# Autodesk Inventor assembly: Upper Lift Limit Switch
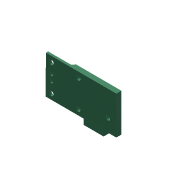
[picture p0: Inventor's stored thumbnail of the model, 180x180]
Saved by Autodesk Inventor 2018 (Build 220112000, 112)
## iProperties
Created: 2018-12-23
Part Number: Upper Lift Limit Switch
Document SubType Name: Assembly
Designer: ball
Author: ball
## Documents named in this file (3)
- C:\FTC\FTC8863CAD\2018Robot\Upper Lift Limit Switch.iam
- C:\FTC\FTC8863CAD\2018Robot\VWheelArmThickRIght.ipt
- C:\FTC\FTC8863CAD\Actobotics\605 parts\605632.ipt
## Components (2 placed, 2 different names)
1. VWheelArmThickRIght:1 — Mate:1, Flush:1, Flush:2
2. 605632:1 — Mate:1, Flush:1, Flush:2
## Relationships (3: Flush 2, Mate 1)
- Mate:1 (6.35 mm): VWheelArmThickRIght:1 ↔ 605632:1
- Flush:1 (12.7 mm): VWheelArmThickRIght:1 ↔ 605632:1
- Flush:2 (33.274 mm): VWheelArmThickRIght:1 ↔ 605632:1
